# Autodesk Inventor assembly: Assembly2
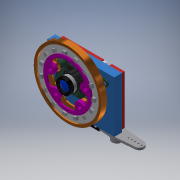
[picture p0: Inventor's stored thumbnail of the model, 180x180]
Saved by Autodesk Inventor 2017 (Build 210142000, 142)
## iProperties
Created: 2016-12-20
Part Number: Assembly2
Document SubType Name: Assembly
Designer: PLTW
Author: PLTW
## Documents named in this file (10)
- C:\Users\margr\OneDrive\Documents\Inventor\Pixy\Assembly2.iam
- C:\Users\margr\OneDrive\Documents\Inventor\Pixy\PixyCamKinda.ipt
- C:\Users\margr\OneDrive\Documents\Inventor\Pixy\focusSpacer.ipt
- C:\Users\margr\OneDrive\Documents\Inventor\Pixy\LEDRing.ipt
- C:\Users\margr\OneDrive\Documents\Inventor\Pixy\backCase.ipt
- C:\Users\margr\OneDrive\Documents\Inventor\Pixy\frontCase.ipt
- C:\Users\margr\OneDrive\Documents\Inventor\Pixy\Ring Front.ipt
- C:\Users\margr\OneDrive\Documents\Inventor\Pixy\Ring Holder.ipt
- C:\Users\margr\OneDrive\Documents\Inventor\Pixy\The Holdy Thing.ipt
- C:\Users\margr\OneDrive\Documents\Inventor\Pixy\servo arm.ipt
## Components (9 placed, 9 different names)
1. PixyCamKinda:1 — Insert:1, Insert:2, Flush:1, Flush:2, Flush:3, Flush:4
2. focusSpacer:1 — Insert:1
3. LEDRing:1 — Insert:2, Flush:6, Flush:7
4. backCase:1 — Flush:1, Flush:2, Flush:5, Mate:1
5. frontCase:1 — Flush:3, Flush:4, Flush:5, Flush:11, Flush:12
6. Ring Front:1 — Flush:6, Flush:7, Flush:8, Flush:9
7. Ring Holder:1 — Flush:8, Flush:9, Flush:10
8. The Holdy Thing:1 — Flush:10, Flush:11, Flush:12
9. servo arm:1 — Mate:1
## Relationships (15: Flush 12, Insert 2, Mate 1)
- Insert:1: PixyCamKinda:1 ↔ focusSpacer:1
- Insert:2: PixyCamKinda:1 ↔ LEDRing:1
- Flush:1: PixyCamKinda:1 ↔ backCase:1
- Flush:2: PixyCamKinda:1 ↔ backCase:1
- Flush:3: PixyCamKinda:1 ↔ frontCase:1
- Flush:4: PixyCamKinda:1 ↔ frontCase:1
- Flush:5: backCase:1 ↔ frontCase:1
- Flush:6: LEDRing:1 ↔ Ring Front:1
- Flush:7: LEDRing:1 ↔ Ring Front:1
- Flush:8: Ring Front:1 ↔ Ring Holder:1
- Flush:9: Ring Front:1 ↔ Ring Holder:1
- Flush:10: Ring Holder:1 ↔ The Holdy Thing:1
- Flush:11: frontCase:1 ↔ The Holdy Thing:1
- Flush:12: frontCase:1 ↔ The Holdy Thing:1
- Mate:1 (6.35 mm): backCase:1 ↔ servo arm:1
